# Autodesk Inventor assembly: mountstestfit
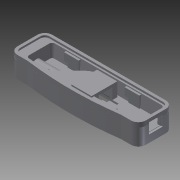
[picture p0: Inventor's stored thumbnail of the model, 180x180]
Saved by Autodesk Inventor 2014 (Build 180170000, 170)
## iProperties
Created: 2014-04-06
Part Number: mountstestfit
Document SubType Name: Assembly
Designer: Tyler
Author: Tyler
## Documents named in this file (3)
- C:\Users\Tyler\Documents\ft8900cad\mountstestfit.iam
- C:\Users\Tyler\Documents\ft8900cad\mount_radio.ipt
- C:\Users\Tyler\Documents\ft8900cad\mount_head.ipt
## Components (2 placed, 2 different names)
1. mount_radio:1 — Flush:1, Flush:2, Mate:1
2. mount_head:1 — Flush:1, Flush:2, Mate:1
## Relationships (3: Flush 2, Mate 1)
- Flush:1: mount_radio:1 ↔ mount_head:1
- Flush:2: mount_radio:1 ↔ mount_head:1
- Mate:1: mount_radio:1 ↔ mount_head:1
